# Autodesk Inventor assembly: motor_w_wheel
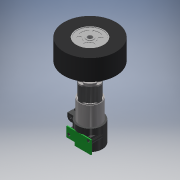
[picture p0: Inventor's stored thumbnail of the model, 180x180]
Saved by Autodesk Inventor 2017 (Build 210142000, 142)
## iProperties
Created: 2016-10-28
Part Number: motor_w_wheel
Document SubType Name: Assembly
Designer: Nick
Sending System: SolidWorks 2016
Last Author: Usuario
Last Saved: 2016-10-28
Author: Nick
## Documents named in this file (6)
- C:\Users\Nick\Desktop\RobotCAD\motor_w_wheel.iam
- C:\Users\Nick\Documents\Inventor\N_1.ipt
- C:\Users\Nick\Documents\Inventor\N_2.ipt
- C:\Users\Nick\Documents\Inventor\N_3.ipt
- C:\Users\Nick\Desktop\RobotCAD\inner_wheel.ipt
- C:\Users\Nick\Desktop\RobotCAD\wheel.ipt
## Components (6 placed, 5 different names)
1. N_1:1 — Mate:5, Mate:6
2. N_2:1 — Mate:3, Mate:5
3. N_3:1
4. inner_wheel:1 — Mate:1, Mate:2, Mate:3, Flush:1, Mate:6
5. inner_wheel:2 — Mate:1, Mate:2, Mate:4
6. wheel:1 — Mate:4, Flush:1
## Relationships (7: Mate 6, Flush 1)
- Mate:1: inner_wheel:1 ↔ inner_wheel:2
- Mate:2: inner_wheel:1 ↔ inner_wheel:2
- Mate:3: N_2:1 ↔ inner_wheel:1
- Mate:4: inner_wheel:2 ↔ wheel:1
- Flush:1: inner_wheel:1 ↔ wheel:1
- Mate:5: N_1:1 ↔ N_2:1
- Mate:6 (10 mm): N_1:1 ↔ inner_wheel:1
